# Autodesk Inventor assembly: 5 Objektivhalterung
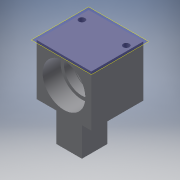
[picture p0: Inventor's stored thumbnail of the model, 180x180]
Saved by Autodesk Inventor 2018.3 (Build 223284000, 284)
## iProperties
Created: 2018-11-29
Part Number: 5 Objektivhalterung
Material: Generisch
Document SubType Name: Assembly
Designer: pgmadmin
Author: pgmadmin
## Documents named in this file (3)
- C:\Users\alexander.steinhoff\Desktop\5 Objektivhalterung.iam
- C:\Users\alexander.steinhoff\Desktop\5 Objektivhalterung oben 29112018.ipt
- C:\Users\alexander.steinhoff\Desktop\5 Objektivhalterung unten 29112018.ipt
## Components (2 placed, 2 different names)
1. 5 Objektivhalterung oben 29112018:1 — Einfügen:1, Passend:1
2. 5 Objektivhalterung unten 29112018:1 — Einfügen:1, Passend:1
## Relationships (2: Insert 1, Mate 1)
- Einfügen:1 [Insert]: 5 Objektivhalterung oben 29112018:1 ↔ 5 Objektivhalterung unten 29112018:1
- Passend:1 [Mate]: 5 Objektivhalterung oben 29112018:1 ↔ 5 Objektivhalterung unten 29112018:1
